# Autodesk Inventor assembly: fork lift
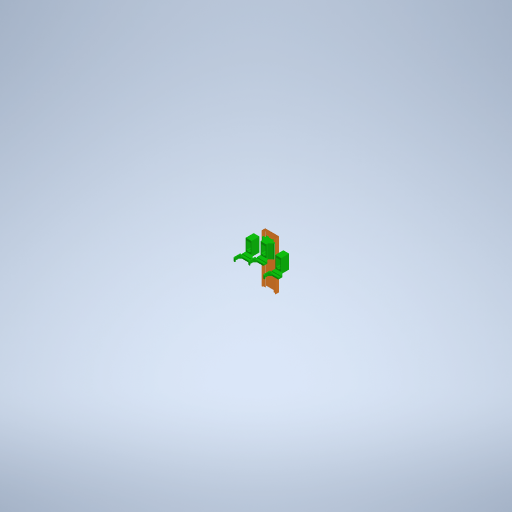
[picture p0: Inventor's stored thumbnail of the model, 512x512]
Saved by Autodesk Inventor 2024 (Build 280153000, 153)
## iProperties
Created: 2024-03-13
Part Number: fork lift
Document SubType Name: Assembly
Designer: dustp
Author: dustp
## Documents named in this file (4)
- C:\Users\dustp\Downloads\robot stuff\fork lift.iam
- C:\Users\dustp\Downloads\robot stuff\aaaaaa 3.ipt
- C:\Users\dustp\Downloads\robot stuff\lift.ipt
- C:\Users\dustp\Downloads\robot stuff\aaaaaa.ipt
## Components (4 placed, 3 different names)
1. aaaaaa 3:1 — Mate:1, Mate:2, Flush:1, Mate:3, Mate:4, Flush:4
2. lift:1 — Mate:1, Mate:2
3. aaaaaa:1 — Flush:2, Mate:3, Flush:3, Flush:4
4. aaaaaa:2 — Flush:1, Flush:2, Mate:4, Flush:3
## Relationships (8: Mate 4, Flush 4)
- Mate:1 (0.1 mm): aaaaaa 3:1 ↔ lift:1
- Mate:2 (0.25 mm): aaaaaa 3:1 ↔ lift:1
- Flush:1 (12.7 mm): aaaaaa 3:1 ↔ aaaaaa:2
- Flush:2: aaaaaa:1 ↔ aaaaaa:2
- Mate:3 (16.5 mm): aaaaaa 3:1 ↔ aaaaaa:1
- Mate:4 (16.85 mm): aaaaaa 3:1 ↔ aaaaaa:2
- Flush:3: aaaaaa:1 ↔ aaaaaa:2
- Flush:4: aaaaaa 3:1 ↔ aaaaaa:1
